# Autodesk Inventor assembly: Lotus_assembly
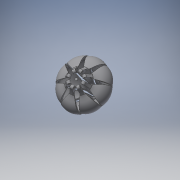
[picture p0: Inventor's stored thumbnail of the model, 180x180]
Saved by Autodesk Inventor 2019 (Build 230136000, 136)
## iProperties
Created: 2019-11-12
Part Number: Lotus_assembly
Document SubType Name: Assembly
Designer: Jorian Brusind
Author: Jorian Brusind
## Documents named in this file (3)
- C:\Users\Jorian Brusind\Documents\GitHub\PersonalProjects\Inventor Projects\Johan\Inventor Files\Lotus_assembly.iam
- C:\Users\Jorian Brusind\Documents\GitHub\PersonalProjects\Inventor Projects\Johan\Inventor Files\Lotus_Petal.ipt
- C:\Users\Jorian Brusind\Documents\GitHub\PersonalProjects\Inventor Projects\Johan\Inventor Files\Ring.ipt
## Components (9 placed, 2 different names)
1. Lotus_Petal:1 — Mate:6, Flush:6
2. Lotus_Petal:2 — Mate:2, Flush:2
3. Lotus_Petal:4 — Mate:4, Flush:4
4. Lotus_Petal:5 — Mate:1, Flush:1
5. Lotus_Petal:6 — Mate:3, Flush:3
6. Lotus_Petal:7 — Mate:5, Flush:5
7. Ring:1 — Mate:1, Flush:1, Mate:2, Flush:2, Mate:3, Flush:3, Mate:4, Flush:4, Mate:5, Flush:5, Mate:6, Flush:6, Mate:7, Flush:7, Mate:8, Flush:8
8. Lotus_Petal:8 — Mate:7, Flush:7
9. Lotus_Petal:9 — Mate:8, Flush:8
## Relationships (16: Mate 8, Flush 8)
- Mate:1: Lotus_Petal:5 ↔ Ring:1
- Flush:1: Lotus_Petal:5 ↔ Ring:1
- Mate:2: Lotus_Petal:2 ↔ Ring:1
- Flush:2: Lotus_Petal:2 ↔ Ring:1
- Mate:3: Lotus_Petal:6 ↔ Ring:1
- Flush:3: Lotus_Petal:6 ↔ Ring:1
- Mate:4: Lotus_Petal:4 ↔ Ring:1
- Flush:4: Lotus_Petal:4 ↔ Ring:1
- Mate:5: Lotus_Petal:7 ↔ Ring:1
- Flush:5: Lotus_Petal:7 ↔ Ring:1
- Mate:6: Lotus_Petal:1 ↔ Ring:1
- Flush:6: Lotus_Petal:1 ↔ Ring:1
- Mate:7: Ring:1 ↔ Lotus_Petal:8
- Flush:7: Ring:1 ↔ Lotus_Petal:8
- Mate:8: Ring:1 ↔ Lotus_Petal:9
- Flush:8: Ring:1 ↔ Lotus_Petal:9
